# Autodesk Inventor assembly: Peli 1300
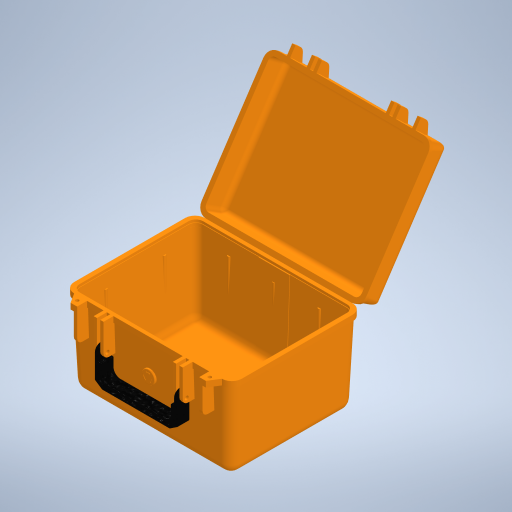
[picture p0: Inventor's stored thumbnail of the model, 512x512]
Saved by Autodesk Inventor 2023.1 (Build 271208000, 208)
## iProperties
Created: 2021-11-22
Part Number: Peli 1300
Description: STEP AP214
Document SubType Name: Assembly
Designer: Charlie Kendall
Sending System: SolidWorks 2018
Preprocessor: SwSTEP 2.0
Title: Peli 1300.STEP
Revision Number: ANY
## Documents named in this file (4)
- C:\Users\Charlie Kendall\Documents\Field Computer\Peli 1300.iam
- C:\Users\Charlie Kendall\Documents\Field Computer\Case and Bezel\1300-CASE-BOT.ipt
- C:\Users\Charlie Kendall\Documents\Field Computer\Case and Bezel\1300-CASE-TOP.ipt
- C:\Users\Charlie Kendall\Documents\Field Computer\Case and Bezel\handle.ipt
## Components (3 placed, 3 different names)
1. 1300-CASE-BOT_1 — Mate:1, Flush:1, Flush:2, Flush:3, Mate:2, Mate:3, Mate:4, Flush:4
2. 1300-CASE-TOP_2 — Mate:4, Flush:4
3. handle_3 — Mate:2, Mate:3
## Relationships (8: Mate 4, Flush 4)
- Mate:1: 1300-CASE-BOT_1
- Flush:1: 1300-CASE-BOT_1
- Flush:2: 1300-CASE-BOT_1
- Flush:3: 1300-CASE-BOT_1
- Mate:2: 1300-CASE-BOT_1 ↔ handle_3
- Mate:3: 1300-CASE-BOT_1 ↔ handle_3
- Mate:4: 1300-CASE-BOT_1 ↔ 1300-CASE-TOP_2
- Flush:4: 1300-CASE-BOT_1 ↔ 1300-CASE-TOP_2
